# Autodesk Inventor assembly: デフォルト底面
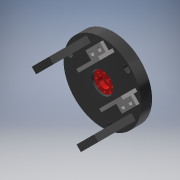
[picture p0: Inventor's stored thumbnail of the model, 180x180]
Saved by Autodesk Inventor 2018 (Build 220112000, 112)
## iProperties
Created: 2018-12-25
Part Number: デフォルト底面
Material: 一般
Document SubType Name: Assembly
Designer: lowyu
Author: lowyu
## Documents named in this file (4)
- C:\Users\lowyu\Desktop\HAND\シャッターハンド\卒論\デフォルト底面.iam
- C:\Users\lowyu\Desktop\HAND\シャッターハンド\モータ固定板3.ipt
- C:\Users\lowyu\Desktop\HAND\シャッターハンド\取付プレート兼　治具.ipt
- C:\Users\lowyu\Desktop\HAND\シャッターハンド\底面 3盆指.ipt
## Components (4 placed, 3 different names)
1. モータ固定板3:1 — メイト:1, メイト:2, メイト:3, メイト:4, メイト:5, メイト:6, メイト:7, メイト:8
2. 取付プレート兼　治具:1 — メイト:4, メイト:5, メイト:6
3. 取付プレート兼　治具:2 — メイト:1, メイト:2, メイト:3
4. 底面 3盆指:1 — メイト:7, メイト:8
## Relationships (8: Mate 8)
- メイト:1 [Mate]: モータ固定板3:1 ↔ 取付プレート兼　治具:2
- メイト:2 [Mate]: モータ固定板3:1 ↔ 取付プレート兼　治具:2
- メイト:3 [Mate]: モータ固定板3:1 ↔ 取付プレート兼　治具:2
- メイト:4 [Mate]: モータ固定板3:1 ↔ 取付プレート兼　治具:1
- メイト:5 [Mate]: モータ固定板3:1 ↔ 取付プレート兼　治具:1
- メイト:6 [Mate]: モータ固定板3:1 ↔ 取付プレート兼　治具:1
- メイト:7 [Mate]: モータ固定板3:1 ↔ 底面 3盆指:1
- メイト:8 [Mate]: モータ固定板3:1 ↔ 底面 3盆指:1
